# Autodesk Inventor assembly: Assembly Macaco
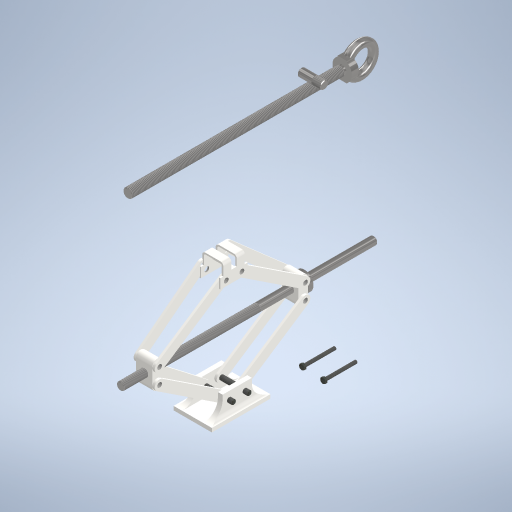
[picture p0: Inventor's stored thumbnail of the model, 512x512]
Saved by Autodesk Inventor 2024 (Build 280153000, 153)
## iProperties
Created: 2024-06-01
Part Number: Assembly Macaco
Document SubType Name: Assembly
Designer: Pedro
d10: 0,000 mm
w_Braço: 12,000 mm
Author: Pedro
## Documents named in this file (18)
- C:\Users\Pedro\Desktop\Autodesk Inbentor\Projeto\Assembly Macaco.iam
- C:\Users\Pedro\Desktop\Autodesk Inbentor\Projeto\Base Macaco.ipt
- C:\Users\Pedro\Desktop\Autodesk Inbentor\Projeto\Braço Macaco.ipt
- C:\Users\Pedro\Desktop\Autodesk Inbentor\Projeto\Junção Fuso.ipt
- C:\Users\Pedro\Desktop\Autodesk Inbentor\Projeto\Encaixe Macaco.ipt
- C:\Users\Pedro\Documents\Inventor\Content Center Files\R2024\en-US\ISO 4018\ISO 4018 - M12 x 90.ipt
- C:\Users\Pedro\Desktop\Autodesk Inbentor\Projeto\DIN 580 - M24 x 600 x 3 x 2.ipt
- C:\Users\Pedro\Documents\Inventor\Content Center Files\R2024\en-US\DIN 427\DIN 427 - M20 x 60.ipt
- C:\Users\Pedro\Documents\Inventor\Content Center Files\R2024\en-US\DIN 615\DIN 615 - E 20 - 20 x 47 x 12.ipt
- C:\Users\Pedro\Desktop\Autodesk Inbentor\Projeto\DIN 427 - M20 x 650.ipt
- C:\Users\Pedro\Documents\Inventor\Content Center Files\R2024\en-US\ISO 4018\ISO 4018 - M8 x 80.ipt
- C:\Users\Pedro\Desktop\Autodesk Inbentor\Projeto\ISO 4018 - M8 x 80.ipt
- C:\Users\Pedro\Desktop\Autodesk Inbentor\Projeto\Assembly Macaco\AIP\FEA\epzg9a0f4.fins
- C:\Users\Pedro\Desktop\Autodesk Inbentor\Projeto\Assembly Macaco\AIP\FEA\epzg9a0g0.fsat
- C:\Users\Pedro\Desktop\Autodesk Inbentor\Projeto\Assembly Macaco\AIP\FEA\epzg9a0g0.ftes
- C:\Users\Pedro\Desktop\Autodesk Inbentor\Projeto\Assembly Macaco\AIP\FEA\epzg9a0g0.fwiz
- C:\Users\Pedro\Desktop\Autodesk Inbentor\Projeto\Assembly Macaco\AIP\FEA\epzg9a0m8.fmsh
- C:\Users\Pedro\Desktop\Autodesk Inbentor\Projeto\Assembly Macaco\AIP\FEA\epzg9a0m9.fres
## Components (20 placed, 11 different names)
1. Base Macaco:1 — Insert:5, Insert:6, Insert:7, Insert:21, Insert:22, Insert:33, Angle:2, Angle:3
2. Braço Macaco:2 — Insert:5, Insert:9
3. Braço Macaco:3 — Insert:6, Insert:10
4. Braço Macaco:4 — Insert:7
5. Junção Fuso:1 — Insert:9, Insert:14, Insert:15, Angle:1, Mate:2, Mate:8
6. Junção Fuso:2 — Insert:10, Angle:1, Angle:2, Mate:2, Mate:4, Mate:6, Mate:7, Insert:41, Insert:42
7. Braço Macaco:5 — Insert:31, Mate:7
8. Braço Macaco:6 — Insert:14, Insert:32
9. Braço Macaco:7 — Mate:6
10. Braço Macaco:8 — Insert:15
11. Encaixe Macaco:1 — Insert:31, Insert:32, Angle:3
12. ISO 4018 M12 x 90:1 — Insert:22
13. ISO 4018 M12 x 90:2 — Insert:21
14. DIN 580 - M24 x 600 x 3 x 2:1
15. Braço Macaco:9 — Insert:33, Mate:4
16. DIN 427 M20 x 60:1
17. DIN 615 E 20 - 20 x 47 x 12:1 — Insert:42
18. DIN 427 - M20 x 650:1 — Insert:41, Mate:8
19. ISO 4018 M8 x 80:1
20. ISO 4018 - M8 x 80:1
## Relationships (22: Insert 14, Mate 5, Angle 3)
- Insert:5: Base Macaco:1 ↔ Braço Macaco:2
- Insert:6: Base Macaco:1 ↔ Braço Macaco:3
- Insert:7: Base Macaco:1 ↔ Braço Macaco:4
- Insert:9: Braço Macaco:2 ↔ Junção Fuso:1
- Insert:10: Braço Macaco:3 ↔ Junção Fuso:2
- Insert:14: Junção Fuso:1 ↔ Braço Macaco:6
- Insert:15: Junção Fuso:1 ↔ Braço Macaco:8
- Insert:21: Base Macaco:1 ↔ ISO 4018 M12 x 90:2
- Insert:22: Base Macaco:1 ↔ ISO 4018 M12 x 90:1
- Insert:31: Braço Macaco:5 ↔ Encaixe Macaco:1
- Insert:32: Braço Macaco:6 ↔ Encaixe Macaco:1
- Insert:33: Base Macaco:1 ↔ Braço Macaco:9
- Angle:1 (180 deg): Junção Fuso:1 ↔ Junção Fuso:2
- Angle:2 (0 deg): Base Macaco:1 ↔ Junção Fuso:2
- Mate:2 (252.272 mm): Junção Fuso:1 ↔ Junção Fuso:2
- Mate:4: Junção Fuso:2 ↔ Braço Macaco:9
- Mate:6: Junção Fuso:2 ↔ Braço Macaco:7
- Mate:7: Junção Fuso:2 ↔ Braço Macaco:5
- Insert:41 (-185 mm): Junção Fuso:2 ↔ DIN 427 - M20 x 650:1
- Mate:8: Junção Fuso:1 ↔ DIN 427 - M20 x 650:1
- Insert:42: Junção Fuso:2 ↔ DIN 615 E 20 - 20 x 47 x 12:1
- Angle:3 (0 deg): Base Macaco:1 ↔ Encaixe Macaco:1
## Named parameters: sa_0 = 1962
note: some values were not read from the file. Shown as the stored number, unit unknown: "sa_0".
